# Autodesk Inventor assembly: FinalRev2
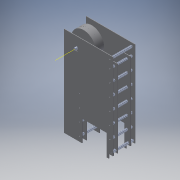
[picture p0: Inventor's stored thumbnail of the model, 180x180]
Saved by Autodesk Inventor 2016 (Build 200138000, 138)
## iProperties
Created: 2017-01-26
Part Number: FinalRev2
Document SubType Name: Assembly
Designer: Nick
Author: Nick
## Documents named in this file (11)
- C:\Users\gagnonc\Documents\GitHub\Robot2017\Assemblies\FinalRev2.iam
- C:\Users\gagnonc\Documents\GitHub\Robot2017\LauncherSidePlateRev2.ipt
- C:\Users\gagnonc\Documents\GitHub\Robot2017\GearboxPlateRev3.ipt
- C:\Users\gagnonc\Documents\GitHub\Robot2017\Parts\3InchChurro.ipt
- C:\Users\gagnonc\Documents\GitHub\Robot2017\Parts\1InchChurro.ipt
- C:\Users\gagnonc\Documents\GitHub\Robot2017\Parts\5,25InchChurro.ipt
- C:\Users\gagnonc\Documents\GitHub\Robot2017\Parts\FlywheelAxle.ipt
- C:\Users\gagnonc\Documents\GitHub\Robot2017\Parts\18TPulley.ipt
- C:\Users\gagnonc\Documents\GitHub\Robot2017\Parts\6InchWheel.ipt
- C:\Users\gagnonc\Documents\GitHub\Robot2017\Parts\FlywheelAxleSpacer.ipt
- C:\Users\gagnonc\Documents\GitHub\Robot2017\Parts\HexShaftCollar.ipt
## Components (47 placed, 10 different names)
1. LauncherSidePlateRev2:1 — Mate:1, Mate:3, Mate:5, Mate:8, Mate:10, Mate:12, Mate:14, Mate:16, Mate:18, Mate:20, Mate:22, Mate:24, Mate:26, Mate:28, Flush:1, Flush:2, Flush:3, Flush:4, Mate:29, Mate:30, Mate:32, Mate:35, Mate:36, Mate:38, Mate:41, Mate:43, Mate:45, Mate:46, Mate:48, Mate:50, Mate:53, Mate:57, Mate:59, Mate:65, Mate:66, Mate:70, Mate:74
2. LauncherSidePlateRev2:2 — Mate:2, Mate:4, Mate:6, Mate:7, Mate:9, Mate:11, Mate:13, Mate:15, Mate:17, Mate:19, Mate:21, Mate:23, Mate:25, Flush:1, Flush:4, Mate:30, Mate:37, Mate:39, Mate:40, Mate:42, Mate:44, Mate:47, Mate:56, Mate:58, Mate:60, Mate:61, Mate:62, Mate:63, Mate:75, Mate:76, Mate:77, Mate:78, Mate:79, Mate:80, Mate:81, Mate:82, Mate:83, Mate:84, Mate:85, Mate:86, Mate:87, Mate:88, Mate:89, Mate:90, Mate:91, Mate:92, Mate:93, Mate:94, Mate:95, Mate:96, Flush:5, Flush:6, Mate:97
3. GearboxPlateRev3:1 — Flush:5, Flush:6, Mate:97, Mate:98
4. GearboxPlateRev3:2 — Mate:26, Mate:27, Flush:2, Flush:3, Mate:31, Mate:33, Mate:49, Mate:51, Mate:52, Mate:54, Mate:55, Mate:64, Mate:67, Mate:68, Mate:69, Mate:72, Mate:73, Flush:7, Mate:99, Mate:100, Flush:8
5. 3InchChurro:1 — Mate:1, Mate:2, Mate:3, Mate:4, Mate:34, Mate:36
6. 3InchChurro:2 — Mate:5, Mate:6, Mate:7, Mate:29, Mate:39
7. 3InchChurro:3 — Mate:8, Mate:9, Mate:40, Mate:41
8. 3InchChurro:4 — Mate:10, Mate:11, Mate:42, Mate:43
9. 3InchChurro:5 — Mate:12, Mate:13, Mate:62, Mate:63
10. 3InchChurro:6 — Mate:14, Mate:15, Mate:44, Mate:47
11. 3InchChurro:7 — Mate:16, Mate:17, Mate:45, Mate:46
12. 3InchChurro:8 — Mate:18, Mate:19, Mate:37, Mate:38
13. 3InchChurro:9 — Mate:22, Mate:23, Mate:58, Mate:59
14. 3InchChurro:10 — Mate:24, Mate:25, Mate:60, Mate:61
15. 3InchChurro:11 — Mate:20, Mate:21, Mate:56, Mate:57
16. 1InchChurro:1 — Mate:27, Mate:28, Mate:31, Mate:32
17. 1InchChurro:2 — Mate:33, Mate:34, Mate:35
18. 1InchChurro:3 — Mate:52, Mate:53
19. 1InchChurro:4 — Mate:54, Mate:55
20. 1InchChurro:5 — Mate:48, Mate:49
21. 1InchChurro:6 — Mate:50, Mate:51
22. 1InchChurro:7 — Mate:64, Mate:65
23. 1InchChurro:9 — Mate:70, Mate:72
24. 1InchChurro:10 — Mate:68, Mate:69
25. 1InchChurro:11 — Mate:66, Mate:67
26. 1InchChurro:12 — Mate:73, Mate:74
27. 1InchChurro:13 — Mate:75, Mate:78
28. 1InchChurro:14 — Mate:76, Mate:77
29. 1InchChurro:15 — Mate:79, Mate:80
30. 1InchChurro:16 — Mate:81, Mate:83
31. 1InchChurro:17 — Mate:82, Mate:84
32. 1InchChurro:18 — Mate:85, Mate:86
33. 1InchChurro:19 — Mate:87, Mate:88
34. 1InchChurro:20 — Mate:91, Mate:96
35. 1InchChurro:21 — Mate:89, Mate:90
36. 1InchChurro:22 — Mate:92, Mate:95
37. 1InchChurro:23 — Mate:93, Mate:94
38. 5,25InchChurro:1 — Mate:98, Mate:99
39. FlywheelAxle:1 — Mate:100, Mate:101, Mate:102, Mate:103, Mate:104, Mate:105, Mate:106, Mate:107, Mate:108, Flush:8
40. 18TPulley:1 — Mate:101, Mate:111, Mate:114
41. 6InchWheel:1 — Mate:102, Mate:109, Mate:110
42. 6InchWheel:2 — Mate:103, Mate:109, Mate:112
43. FlywheelAxleSpacer:1 — Mate:104, Mate:110, Mate:111
44. FlywheelAxleSpacer:2 — Mate:106, Mate:113, Mate:115
45. FlywheelAxleSpacer:3 — Mate:105, Mate:112, Mate:113
46. HexShaftCollar:1 — Mate:108, Mate:114
47. HexShaftCollar:2 — Mate:107, Mate:115
## Relationships (122: Mate 114, Flush 8)
- Mate:1: LauncherSidePlateRev2:1 ↔ 3InchChurro:1
- Mate:2: LauncherSidePlateRev2:2 ↔ 3InchChurro:1
- Mate:3: LauncherSidePlateRev2:1 ↔ 3InchChurro:1
- Mate:4: LauncherSidePlateRev2:2 ↔ 3InchChurro:1
- Mate:5: LauncherSidePlateRev2:1 ↔ 3InchChurro:2
- Mate:6: LauncherSidePlateRev2:2 ↔ 3InchChurro:2
- Mate:7: LauncherSidePlateRev2:2 ↔ 3InchChurro:2
- Mate:8: LauncherSidePlateRev2:1 ↔ 3InchChurro:3
- Mate:9: LauncherSidePlateRev2:2 ↔ 3InchChurro:3
- Mate:10: LauncherSidePlateRev2:1 ↔ 3InchChurro:4
- Mate:11: LauncherSidePlateRev2:2 ↔ 3InchChurro:4
- Mate:12: LauncherSidePlateRev2:1 ↔ 3InchChurro:5
- Mate:13: LauncherSidePlateRev2:2 ↔ 3InchChurro:5
- Mate:14: LauncherSidePlateRev2:1 ↔ 3InchChurro:6
- Mate:15: LauncherSidePlateRev2:2 ↔ 3InchChurro:6
- Mate:16: LauncherSidePlateRev2:1 ↔ 3InchChurro:7
- Mate:17: LauncherSidePlateRev2:2 ↔ 3InchChurro:7
- Mate:18: LauncherSidePlateRev2:1 ↔ 3InchChurro:8
- Mate:19: LauncherSidePlateRev2:2 ↔ 3InchChurro:8
- Mate:20: LauncherSidePlateRev2:1 ↔ 3InchChurro:11
- Mate:21: LauncherSidePlateRev2:2 ↔ 3InchChurro:11
- Mate:22: LauncherSidePlateRev2:1 ↔ 3InchChurro:9
- Mate:23: LauncherSidePlateRev2:2 ↔ 3InchChurro:9
- Mate:24: LauncherSidePlateRev2:1 ↔ 3InchChurro:10
- Mate:25: LauncherSidePlateRev2:2 ↔ 3InchChurro:10
- Mate:26: LauncherSidePlateRev2:1 ↔ GearboxPlateRev3:2
- Mate:27: GearboxPlateRev3:2 ↔ 1InchChurro:1
- Mate:28: LauncherSidePlateRev2:1 ↔ 1InchChurro:1
- Flush:1: LauncherSidePlateRev2:1 ↔ LauncherSidePlateRev2:2
- Flush:2: LauncherSidePlateRev2:1 ↔ GearboxPlateRev3:2
- Flush:3: LauncherSidePlateRev2:1 ↔ GearboxPlateRev3:2
- Flush:4: LauncherSidePlateRev2:1 ↔ LauncherSidePlateRev2:2
- Mate:29: LauncherSidePlateRev2:1 ↔ 3InchChurro:2
- Mate:30 (76.2 mm): LauncherSidePlateRev2:1 ↔ LauncherSidePlateRev2:2
- Mate:31: GearboxPlateRev3:2 ↔ 1InchChurro:1
- Mate:32: LauncherSidePlateRev2:1 ↔ 1InchChurro:1
- Mate:33: GearboxPlateRev3:2 ↔ 1InchChurro:2
- Mate:34: 3InchChurro:1 ↔ 1InchChurro:2
- Mate:35: LauncherSidePlateRev2:1 ↔ 1InchChurro:2
- Mate:36: LauncherSidePlateRev2:1 ↔ 3InchChurro:1
- Mate:37: LauncherSidePlateRev2:2 ↔ 3InchChurro:8
- Mate:38: LauncherSidePlateRev2:1 ↔ 3InchChurro:8
- Mate:39: LauncherSidePlateRev2:2 ↔ 3InchChurro:2
- Mate:40: LauncherSidePlateRev2:2 ↔ 3InchChurro:3
- Mate:41: LauncherSidePlateRev2:1 ↔ 3InchChurro:3
- Mate:42: LauncherSidePlateRev2:2 ↔ 3InchChurro:4
- Mate:43: LauncherSidePlateRev2:1 ↔ 3InchChurro:4
- Mate:44: LauncherSidePlateRev2:2 ↔ 3InchChurro:6
- Mate:45: LauncherSidePlateRev2:1 ↔ 3InchChurro:7
- Mate:46: LauncherSidePlateRev2:1 ↔ 3InchChurro:7
- Mate:47: LauncherSidePlateRev2:2 ↔ 3InchChurro:6
- Mate:48: LauncherSidePlateRev2:1 ↔ 1InchChurro:5
- Mate:49: GearboxPlateRev3:2 ↔ 1InchChurro:5
- Mate:50: LauncherSidePlateRev2:1 ↔ 1InchChurro:6
- Mate:51: GearboxPlateRev3:2 ↔ 1InchChurro:6
- Mate:52: GearboxPlateRev3:2 ↔ 1InchChurro:3
- Mate:53: LauncherSidePlateRev2:1 ↔ 1InchChurro:3
- Mate:54: GearboxPlateRev3:2 ↔ 1InchChurro:4
- Mate:55: GearboxPlateRev3:2 ↔ 1InchChurro:4
- Mate:56: LauncherSidePlateRev2:2 ↔ 3InchChurro:11
- Mate:57: LauncherSidePlateRev2:1 ↔ 3InchChurro:11
- Mate:58: LauncherSidePlateRev2:2 ↔ 3InchChurro:9
- Mate:59: LauncherSidePlateRev2:1 ↔ 3InchChurro:9
- Mate:60: LauncherSidePlateRev2:2 ↔ 3InchChurro:10
- Mate:61: LauncherSidePlateRev2:2 ↔ 3InchChurro:10
- Mate:62: LauncherSidePlateRev2:2 ↔ 3InchChurro:5
- Mate:63: LauncherSidePlateRev2:2 ↔ 3InchChurro:5
- Mate:64: GearboxPlateRev3:2 ↔ 1InchChurro:7
- Mate:65: LauncherSidePlateRev2:1 ↔ 1InchChurro:7
- Mate:66: LauncherSidePlateRev2:1 ↔ 1InchChurro:11
- Mate:67: GearboxPlateRev3:2 ↔ 1InchChurro:11
- Mate:68: GearboxPlateRev3:2 ↔ 1InchChurro:10
- Mate:69: GearboxPlateRev3:2 ↔ 1InchChurro:10
- Mate:70: LauncherSidePlateRev2:1 ↔ 1InchChurro:9
- Mate:72: GearboxPlateRev3:2 ↔ 1InchChurro:9
- Mate:73: GearboxPlateRev3:2 ↔ 1InchChurro:12
- Mate:74: LauncherSidePlateRev2:1 ↔ 1InchChurro:12
- Mate:75: LauncherSidePlateRev2:2 ↔ 1InchChurro:13
- Mate:76: LauncherSidePlateRev2:2 ↔ 1InchChurro:14
- Mate:77: LauncherSidePlateRev2:2 ↔ 1InchChurro:14
- Mate:78: LauncherSidePlateRev2:2 ↔ 1InchChurro:13
- Mate:79: LauncherSidePlateRev2:2 ↔ 1InchChurro:15
- Mate:80: LauncherSidePlateRev2:2 ↔ 1InchChurro:15
- Mate:81: LauncherSidePlateRev2:2 ↔ 1InchChurro:16
- Mate:82: LauncherSidePlateRev2:2 ↔ 1InchChurro:17
- Mate:83: LauncherSidePlateRev2:2 ↔ 1InchChurro:16
- Mate:84: LauncherSidePlateRev2:2 ↔ 1InchChurro:17
- Mate:85: LauncherSidePlateRev2:2 ↔ 1InchChurro:18
- Mate:86: LauncherSidePlateRev2:2 ↔ 1InchChurro:18
- Mate:87: LauncherSidePlateRev2:2 ↔ 1InchChurro:19
- Mate:88: LauncherSidePlateRev2:2 ↔ 1InchChurro:19
- Mate:89: LauncherSidePlateRev2:2 ↔ 1InchChurro:21
- Mate:90: LauncherSidePlateRev2:2 ↔ 1InchChurro:21
- Mate:91: LauncherSidePlateRev2:2 ↔ 1InchChurro:20
- Mate:92: LauncherSidePlateRev2:2 ↔ 1InchChurro:22
- Mate:93: LauncherSidePlateRev2:2 ↔ 1InchChurro:23
- Mate:94: LauncherSidePlateRev2:2 ↔ 1InchChurro:23
- Mate:95: LauncherSidePlateRev2:2 ↔ 1InchChurro:22
- Mate:96: LauncherSidePlateRev2:2 ↔ 1InchChurro:20
- Flush:5: LauncherSidePlateRev2:2 ↔ GearboxPlateRev3:1
- Flush:6: LauncherSidePlateRev2:2 ↔ GearboxPlateRev3:1
- Mate:97 (25.4 mm): LauncherSidePlateRev2:2 ↔ GearboxPlateRev3:1
- Flush:7: GearboxPlateRev3:2
- Mate:98: GearboxPlateRev3:1 ↔ 5,25InchChurro:1
- Mate:99: GearboxPlateRev3:2 ↔ 5,25InchChurro:1
- Mate:100: GearboxPlateRev3:2 ↔ FlywheelAxle:1
- Mate:101: FlywheelAxle:1 ↔ 18TPulley:1
- Mate:102: FlywheelAxle:1 ↔ 6InchWheel:1
- Mate:103: FlywheelAxle:1 ↔ 6InchWheel:2
- Mate:104: FlywheelAxle:1 ↔ FlywheelAxleSpacer:1
- Mate:105: FlywheelAxle:1 ↔ FlywheelAxleSpacer:3
- Mate:106: FlywheelAxle:1 ↔ FlywheelAxleSpacer:2
- Mate:107: FlywheelAxle:1 ↔ HexShaftCollar:2
- Mate:108: FlywheelAxle:1 ↔ HexShaftCollar:1
- Mate:109: 6InchWheel:1 ↔ 6InchWheel:2
- Mate:110: 6InchWheel:1 ↔ FlywheelAxleSpacer:1
- Mate:111: 18TPulley:1 ↔ FlywheelAxleSpacer:1
- Mate:112: 6InchWheel:2 ↔ FlywheelAxleSpacer:3
- Mate:113: FlywheelAxleSpacer:2 ↔ FlywheelAxleSpacer:3
- Mate:114: 18TPulley:1 ↔ HexShaftCollar:1
- Mate:115: FlywheelAxleSpacer:2 ↔ HexShaftCollar:2
- Flush:8 (-9.525 mm): GearboxPlateRev3:2 ↔ FlywheelAxle:1
